# Autodesk Inventor assembly: Base Ensamblada
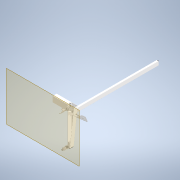
[picture p0: Inventor's stored thumbnail of the model, 180x180]
Saved by Autodesk Inventor 2021.2 (Build 252289000, 289)
## iProperties
Created: 2026-06-02
Part Number: Base Ensamblada
Document SubType Name: Assembly
Designer: nelso
Author: nelso
## Documents named in this file (16)
- C:\Users\nelso\Desktop\Soporte paciente espinografia\Soporte Paciente Espinografia\Workspaces\Workspace\Base Ensamblada.iam
- C:\Users\nelso\Desktop\Soporte paciente espinografia\Soporte Paciente Espinografia\Workspaces\Workspace\tubo1-40x40x1800.ipt
- C:\Users\nelso\Desktop\Soporte paciente espinografia\Soporte Paciente Espinografia\Workspaces\Workspace\tubo2-40x40x1800.ipt
- C:\Users\nelso\Desktop\Soporte paciente espinografia\Soporte Paciente Espinografia\Workspaces\Workspace\tubo1-40x40x640.ipt
- C:\Users\nelso\Desktop\Soporte paciente espinografia\Soporte Paciente Espinografia\Workspaces\Workspace\tubo2-40x40x640.ipt
- C:\Users\nelso\Desktop\Soporte paciente espinografia\Soporte Paciente Espinografia\Workspaces\Workspace\bosch_3842547836_6u5hvyo05ag2294jqeen4vb8k1.iam
- C:\Users\nelso\Desktop\Soporte paciente espinografia\Soporte Paciente Espinografia\Workspaces\Workspace\Cobertora Derecha.ipt
- C:\Users\nelso\Desktop\Soporte paciente espinografia\Soporte Paciente Espinografia\Workspaces\Workspace\Cobertora Izquierda.ipt
- C:\Users\nelso\Desktop\Soporte paciente espinografia\Soporte Paciente Espinografia\Workspaces\Workspace\tubo3-40x80x800.ipt
- C:\Users\nelso\Desktop\Soporte paciente espinografia\Soporte Paciente Espinografia\Workspaces\Workspace\Tapacanto delantero.ipt
- C:\Users\nelso\Desktop\Soporte paciente espinografia\Soporte Paciente Espinografia\Workspaces\Workspace\Tapacanto Superior.ipt
- C:\Users\nelso\Desktop\Soporte paciente espinografia\Soporte Paciente Espinografia\Workspaces\Workspace\RFPLUS8PO300.ipt
- C:\Users\nelso\Desktop\Soporte paciente espinografia\Soporte Paciente Espinografia\Workspaces\Workspace\varilla.ipt
- C:\Users\nelso\Desktop\Soporte paciente espinografia\Soporte Paciente Espinografia\Workspaces\Workspace\buje.ipt
- C:\Users\nelso\Desktop\Soporte paciente espinografia\Soporte Paciente Espinografia\Workspaces\Workspace\pedal.ipt
- C:\Users\nelso\Desktop\Soporte paciente espinografia\Soporte Paciente Espinografia\Workspaces\Workspace\Assembly3.iam
## Components (40 placed, 15 different names)
1. tubo1-40x40x1800:1 — Nivelación:20, Coincidencia:56, Coincidencia:57, Nivelación:30, Coincidencia:69, Coincidencia:70, Nivelación:66, Flush:68, Flush:69, Mate:82, Mate:83, Flush:70, Flush:71, Flush:72, Flush:73, Mate:90, Mate:91, Mate:92, Mate:93
2. tubo2-40x40x1800:1 — Nivelación:17, Coincidencia:54, Coincidencia:55, Coincidencia:68, Nivelación:67, Coincidencia:71, Flush:75, Flush:76, Flush:77, Flush:78, Flush:79, Mate:84, Mate:85, Mate:86, Mate:87, Mate:88, Mate:107, Flush:101
3. tubo1-40x40x640:1 — Mate:14, Coincidencia:27, Nivelación:16, Coincidencia:44, Coincidencia:61, Nivelación:65, Coincidencia:67
4. tubo2-40x40x640:1 — Mate:15, Nivelación:14, Coincidencia:24, Coincidencia:30, Coincidencia:42, Coincidencia:60, Coincidencia:62, Coincidencia:63
5. bosch_3842547836_6u5hvyo05ag2294jqeen4vb8k1:1 [sub-assembly] — Coincidencia:48, Coincidencia:49
6. bosch_3842547836_6u5hvyo05ag2294jqeen4vb8k1:2 [sub-assembly] — Mate:14
7. bosch_3842547836_6u5hvyo05ag2294jqeen4vb8k1:3 [sub-assembly] — Coincidencia:40, Coincidencia:41
8. bosch_3842547836_6u5hvyo05ag2294jqeen4vb8k1:4 [sub-assembly] — Mate:15, Coincidencia:30
9. Cobertora Derecha:1 — Nivelación:14, Coincidencia:24, Nivelación:17, Coincidencia:37, Coincidencia:38, Nivelación:18, Coincidencia:42, Nivelación:26, Coincidencia:55, Nivelación:27, Coincidencia:66, Flush:97, Flush:98, Mate:96, Mate:97
10. Cobertora Izquierda:1 — Coincidencia:27, Nivelación:16, Nivelación:18, Nivelación:20, Coincidencia:44, Coincidencia:50, Coincidencia:51, Nivelación:24, Coincidencia:53, Coincidencia:57, Nivelación:28, Coincidencia:65, Flush:95, Flush:96, Mate:94, Mate:95, Mate:115
11. tubo2-40x40x640:2 — Coincidencia:37, Coincidencia:38, Coincidencia:40, Coincidencia:41, Coincidencia:66
12. tubo2-40x40x640:3 — Coincidencia:48, Coincidencia:49, Coincidencia:50, Coincidencia:51, Coincidencia:65
13. tubo3-40x80x800:1 — Nivelación:24, Nivelación:25, Coincidencia:54, Coincidencia:56, Nivelación:27, Nivelación:28, Mate:110, Mate:111
14. Tapacanto delantero:1 — Coincidencia:60, Coincidencia:62, Coincidencia:63
15. Tapacanto delantero:2 — Coincidencia:61, Nivelación:65, Coincidencia:67
16. Tapacanto Superior:1 — Coincidencia:68, Nivelación:67, Coincidencia:71
17. Tapacanto Superior:2 — Coincidencia:69, Coincidencia:70, Nivelación:66
18. RFPLUS8PO300:1 — Mate:107, Flush:101
19. RFPLUS8PO300:2 — Flush:75, Mate:88
20. RFPLUS8PO300:3 — Flush:76, Mate:87
21. RFPLUS8PO300:4 — Flush:77, Mate:86
22. RFPLUS8PO300:5 — Flush:78, Mate:84
23. RFPLUS8PO300:6 — Flush:79, Mate:85
24. RFPLUS8PO300:7 — Flush:72, Mate:92
25. RFPLUS8PO300:8 — Flush:73, Mate:93
26. RFPLUS8PO300:9 — Flush:70, Mate:90
27. RFPLUS8PO300:10 — Flush:71, Mate:91
28. RFPLUS8PO300:11 — Flush:68, Mate:82
29. RFPLUS8PO300:12 — Flush:69, Mate:83
30. RFPLUS8PO300:13 — Flush:95, Mate:94
31. RFPLUS8PO300:14 — Flush:96, Mate:95
32. RFPLUS8PO300:15 — Flush:97, Mate:97
33. RFPLUS8PO300:16 — Flush:98, Mate:96
34. varilla:1 — Flush:102, Angle:1, Angle:2
35. buje:1 — Mate:116
36. buje:2 — Mate:114, Mate:115, Mate:116
37. pedal:1 — Angle:2
38. pedal:2 — Angle:1
39. Assembly3:1 [sub-assembly] — Mate:110, Mate:114, Flush:103
40. Assembly3:2 [sub-assembly] — Mate:111, Flush:103
## Relationships (87: Mate 53, Flush 32, Angle 2)
- [Mate]: tubo1-40x40x640:1 ↔ bosch_3842547836_6u5hvyo05ag2294jqeen4vb8k1:2
- Mate:14: tubo1-40x40x640:1 ↔ bosch_3842547836_6u5hvyo05ag2294jqeen4vb8k1:2
- Mate:15: tubo2-40x40x640:1 ↔ bosch_3842547836_6u5hvyo05ag2294jqeen4vb8k1:4
- Nivelación:14 [Flush]: tubo2-40x40x640:1 ↔ Cobertora Derecha:1
- Coincidencia:24 [Mate] (0.5 mm): tubo2-40x40x640:1 ↔ Cobertora Derecha:1
- Coincidencia:27 [Mate] (0.5 mm): tubo1-40x40x640:1 ↔ Cobertora Izquierda:1
- Nivelación:16 [Flush]: tubo1-40x40x640:1 ↔ Cobertora Izquierda:1
- Coincidencia:30 [Mate]: tubo2-40x40x640:1 ↔ bosch_3842547836_6u5hvyo05ag2294jqeen4vb8k1:4
- Nivelación:17 [Flush]: tubo2-40x40x1800:1 ↔ Cobertora Derecha:1
- Coincidencia:37 [Mate]: Cobertora Derecha:1 ↔ tubo2-40x40x640:2
- Coincidencia:38 [Mate]: Cobertora Derecha:1 ↔ tubo2-40x40x640:2
- Coincidencia:40 [Mate]: bosch_3842547836_6u5hvyo05ag2294jqeen4vb8k1:3 ↔ tubo2-40x40x640:2
- Coincidencia:41 [Mate]: bosch_3842547836_6u5hvyo05ag2294jqeen4vb8k1:3 ↔ tubo2-40x40x640:2
- Nivelación:18 [Flush]: Cobertora Derecha:1 ↔ Cobertora Izquierda:1
- Coincidencia:42 [Mate]: tubo2-40x40x640:1 ↔ Cobertora Derecha:1
- Nivelación:20 [Flush]: tubo1-40x40x1800:1 ↔ Cobertora Izquierda:1
- Coincidencia:44 [Mate]: tubo1-40x40x640:1 ↔ Cobertora Izquierda:1
- Coincidencia:48 [Mate]: bosch_3842547836_6u5hvyo05ag2294jqeen4vb8k1:1 ↔ tubo2-40x40x640:3
- Coincidencia:49 [Mate]: bosch_3842547836_6u5hvyo05ag2294jqeen4vb8k1:1 ↔ tubo2-40x40x640:3
- Coincidencia:50 [Mate]: Cobertora Izquierda:1 ↔ tubo2-40x40x640:3
- Coincidencia:51 [Mate]: Cobertora Izquierda:1 ↔ tubo2-40x40x640:3
- Nivelación:24 [Flush]: Cobertora Izquierda:1 ↔ tubo3-40x80x800:1
- Nivelación:25 [Flush]: tubo3-40x80x800:1
- Coincidencia:53 [Mate] (395 mm): Cobertora Izquierda:1
- Nivelación:26 [Flush] (395 mm): Cobertora Derecha:1
- Coincidencia:54 [Mate]: tubo2-40x40x1800:1 ↔ tubo3-40x80x800:1
- Coincidencia:55 [Mate]: tubo2-40x40x1800:1 ↔ Cobertora Derecha:1
- Coincidencia:56 [Mate]: tubo1-40x40x1800:1 ↔ tubo3-40x80x800:1
- Coincidencia:57 [Mate]: tubo1-40x40x1800:1 ↔ Cobertora Izquierda:1
- Nivelación:27 [Flush]: Cobertora Derecha:1 ↔ tubo3-40x80x800:1
- Nivelación:28 [Flush]: Cobertora Izquierda:1 ↔ tubo3-40x80x800:1
- Coincidencia:60 [Mate]: tubo2-40x40x640:1 ↔ Tapacanto delantero:1
- Coincidencia:61 [Mate]: tubo1-40x40x640:1 ↔ Tapacanto delantero:2
- Coincidencia:62 [Mate]: tubo2-40x40x640:1 ↔ Tapacanto delantero:1
- Coincidencia:63 [Mate]: tubo2-40x40x640:1 ↔ Tapacanto delantero:1
- Nivelación:65 [Flush]: tubo1-40x40x640:1 ↔ Tapacanto delantero:2
- Coincidencia:67 [Mate]: tubo1-40x40x640:1 ↔ Tapacanto delantero:2
- Coincidencia:65 [Mate]: Cobertora Izquierda:1 ↔ tubo2-40x40x640:3
- Coincidencia:66 [Mate]: Cobertora Derecha:1 ↔ tubo2-40x40x640:2
- Nivelación:30 [Flush]: tubo1-40x40x1800:1
- Coincidencia:68 [Mate]: tubo2-40x40x1800:1 ↔ Tapacanto Superior:1
- Coincidencia:69 [Mate]: tubo1-40x40x1800:1 ↔ Tapacanto Superior:2
- Coincidencia:70 [Mate]: tubo1-40x40x1800:1 ↔ Tapacanto Superior:2
- Nivelación:66 [Flush]: tubo1-40x40x1800:1 ↔ Tapacanto Superior:2
- Nivelación:67 [Flush]: tubo2-40x40x1800:1 ↔ Tapacanto Superior:1
- Coincidencia:71 [Mate]: tubo2-40x40x1800:1 ↔ Tapacanto Superior:1
- Flush:68: tubo1-40x40x1800:1 ↔ RFPLUS8PO300:11
- Flush:69: tubo1-40x40x1800:1 ↔ RFPLUS8PO300:12
- Mate:82: tubo1-40x40x1800:1 ↔ RFPLUS8PO300:11
- Mate:83: tubo1-40x40x1800:1 ↔ RFPLUS8PO300:12
- Flush:70: tubo1-40x40x1800:1 ↔ RFPLUS8PO300:9
- Flush:71: tubo1-40x40x1800:1 ↔ RFPLUS8PO300:10
- Flush:72: tubo1-40x40x1800:1 ↔ RFPLUS8PO300:7
- Flush:73: tubo1-40x40x1800:1 ↔ RFPLUS8PO300:8
- Flush:75: tubo2-40x40x1800:1 ↔ RFPLUS8PO300:2
- Flush:76: tubo2-40x40x1800:1 ↔ RFPLUS8PO300:3
- Flush:77: tubo2-40x40x1800:1 ↔ RFPLUS8PO300:4
- Flush:78: tubo2-40x40x1800:1 ↔ RFPLUS8PO300:5
- Flush:79: tubo2-40x40x1800:1 ↔ RFPLUS8PO300:6
- Mate:84: tubo2-40x40x1800:1 ↔ RFPLUS8PO300:5
- Mate:85: tubo2-40x40x1800:1 ↔ RFPLUS8PO300:6
- Mate:86: tubo2-40x40x1800:1 ↔ RFPLUS8PO300:4
- Mate:87: tubo2-40x40x1800:1 ↔ RFPLUS8PO300:3
- Mate:88: tubo2-40x40x1800:1 ↔ RFPLUS8PO300:2
- Mate:90: tubo1-40x40x1800:1 ↔ RFPLUS8PO300:9
- Mate:91: tubo1-40x40x1800:1 ↔ RFPLUS8PO300:10
- Mate:92: tubo1-40x40x1800:1 ↔ RFPLUS8PO300:7
- Mate:93: tubo1-40x40x1800:1 ↔ RFPLUS8PO300:8
- Flush:95: Cobertora Izquierda:1 ↔ RFPLUS8PO300:13
- Flush:96: Cobertora Izquierda:1 ↔ RFPLUS8PO300:14
- Mate:94: Cobertora Izquierda:1 ↔ RFPLUS8PO300:13
- Mate:95: Cobertora Izquierda:1 ↔ RFPLUS8PO300:14
- Flush:97: Cobertora Derecha:1 ↔ RFPLUS8PO300:15
- Flush:98: Cobertora Derecha:1 ↔ RFPLUS8PO300:16
- Mate:96: Cobertora Derecha:1 ↔ RFPLUS8PO300:16
- Mate:97: Cobertora Derecha:1 ↔ RFPLUS8PO300:15
- Mate:107: tubo2-40x40x1800:1 ↔ RFPLUS8PO300:1
- Flush:101: tubo2-40x40x1800:1 ↔ RFPLUS8PO300:1
- Flush:102: varilla:1
- Angle:1 (0 deg): varilla:1 ↔ pedal:2
- Angle:2 (0 deg): varilla:1 ↔ pedal:1
- Mate:110: tubo3-40x80x800:1 ↔ Assembly3:1
- Mate:111: tubo3-40x80x800:1 ↔ Assembly3:2
- Mate:114: buje:2 ↔ Assembly3:1
- Mate:115: Cobertora Izquierda:1 ↔ buje:2
- Mate:116: buje:1 ↔ buje:2
- Flush:103: Assembly3:1 ↔ Assembly3:2
